# Autodesk Inventor assembly: nc_nhk24
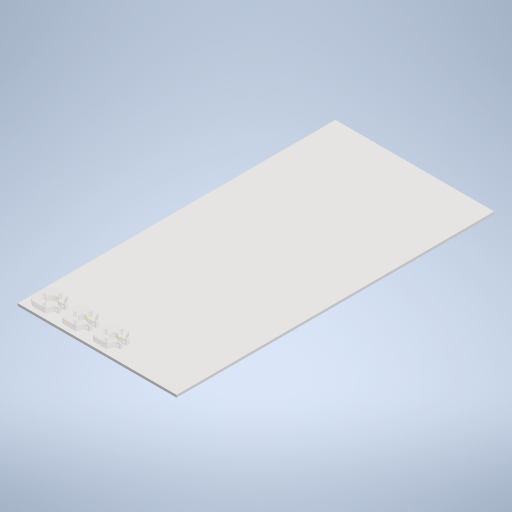
[picture p0: Inventor's stored thumbnail of the model, 512x512]
Saved by Autodesk Inventor 2023 (Build 270158000, 158)
## iProperties
Created: 2022-04-30
Part Number: nc_nhk24
Document SubType Name: Assembly
Designer: yuta
Author: yuta
## Documents named in this file (5)
- C:\Users\yuta\Documents\NHK\nc_nhk24.iam
- C:\Users\yuta\Documents\NHK\NC.port.ipt
- C:\Users\yuta\Documents\NHK\射出_腕固定.ipt
- C:\Users\yuta\Documents\NHK\射出_腕固定2_真.ipt
- C:\Users\yuta\Documents\NHK\射出_腕固定3_真.ipt
## Components (4 placed, 4 different names)
1. NC.port:1 — メイト:1, フラッシュ:1, メイト:2, メイト:3, フラッシュ:2, メイト:5, フラッシュ:3
2. 射出_腕固定:1 — メイト:1, フラッシュ:1, メイト:2, メイト:4
3. 射出_腕固定2_真:1 — メイト:3, フラッシュ:2, メイト:4, メイト:6
4. 射出_腕固定3_真:1 — メイト:5, フラッシュ:3, メイト:6
## Relationships (9: Mate 6, Flush 3)
- メイト:1 [Mate]: NC.port:1 ↔ 射出_腕固定:1
- フラッシュ:1 [Flush] (6 mm): NC.port:1 ↔ 射出_腕固定:1
- メイト:2 [Mate] (-23 mm): NC.port:1 ↔ 射出_腕固定:1
- メイト:3 [Mate]: NC.port:1 ↔ 射出_腕固定2_真:1
- フラッシュ:2 [Flush] (6 mm): NC.port:1 ↔ 射出_腕固定2_真:1
- メイト:4 [Mate] (24 mm): 射出_腕固定:1 ↔ 射出_腕固定2_真:1
- メイト:5 [Mate]: NC.port:1 ↔ 射出_腕固定3_真:1
- フラッシュ:3 [Flush] (6 mm): NC.port:1 ↔ 射出_腕固定3_真:1
- メイト:6 [Mate] (24 mm): 射出_腕固定2_真:1 ↔ 射出_腕固定3_真:1
